# Autodesk Inventor assembly: Lock assembly
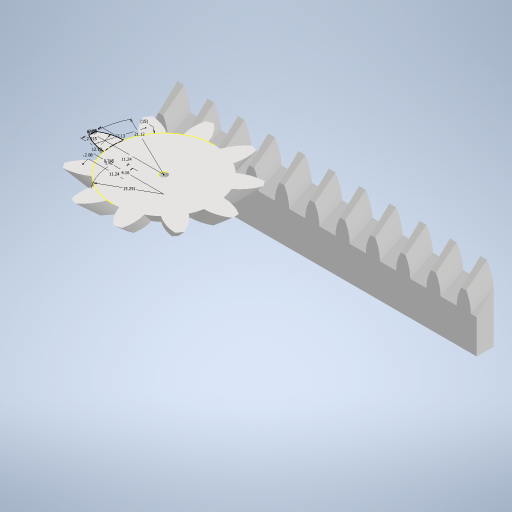
[picture p0: Inventor's stored thumbnail of the model, 512x512]
Saved by Autodesk Inventor 2023 (Build 270158000, 158)
## iProperties
Created: 2022-11-18
Part Number: Lock assembly
Document SubType Name: Assembly
Designer: shrey
Author: shrey
## Documents named in this file (3)
- D:\Inventor Projects\Door Lock\Lock assembly.iam
- D:\Inventor Projects\Door Lock\lockPin.ipt
- D:\Inventor Projects\Door Lock\bevelGear.ipt
## Components (2 placed, 2 different names)
1. lockPin:1 — Rotation/Translation:1
2. bevelGear:1 — Rotation/Translation:1
## Relationships (1: RelateRotateTranslate 1)
- Rotation/Translation:1 [RelateRotateTranslate] (25.4 mm): lockPin:1 ↔ bevelGear:1
